# Autodesk Inventor assembly: A2017_T5_08
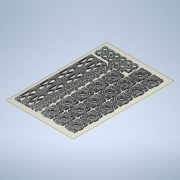
[picture p0: Inventor's stored thumbnail of the model, 180x180]
Saved by Autodesk Inventor 2022 (Build 260153000, 153)
## iProperties
Created: 2022-09-28
Part Number: A2017_T5_08
Document SubType Name: Assembly
Designer: Masato
Author: Masato
## Documents named in this file (6)
- C:\Users\ヨコオリク\Documents\CITBrains\SUSTAINA-OP\Cam\A2017_T5\A2017_T5_08.iam
- C:\Users\ヨコオリク\Documents\CITBrains\SUSTAINA-OP\Cam\DisposableBoard.ipt
- C:\Users\ヨコオリク\Documents\CITBrains\SUSTAINA-OP\UpperBody\UpperBody_horn_frame.ipt
- C:\Users\ヨコオリク\Documents\CITBrains\SUSTAINA-OP\LowerBody\Foot\Foot_root_block.ipt
- C:\Users\ヨコオリク\Documents\CITBrains\SUSTAINA-OP\LowerBody\Knee\Knee_clamp.ipt
- C:\Users\ヨコオリク\Documents\CITBrains\SUSTAINA-OP\LowerBody\Link\BackLink_diagonal.ipt
## Components (61 placed, 5 different names)
1. DisposableBoard:1 — フラッシュ:1, フラッシュ:2, フラッシュ:3, フラッシュ:4, Flush:5, 正接:1, フラッシュ:8, フラッシュ:9, フラッシュ:10, フラッシュ:11, 正接:6
2. Foot_root_block:33 — メイト:14, メイト:15, メイト:16
3. UpperBody_horn_frame:1 — Mate:3, Flush:5, 正接:5
4. UpperBody_horn_frame:2
5. UpperBody_horn_frame:3
6. UpperBody_horn_frame:4
7. UpperBody_horn_frame:5
8. UpperBody_horn_frame:6
9. UpperBody_horn_frame:7 — 正接:1
10. UpperBody_horn_frame:8
11. UpperBody_horn_frame:9
12. UpperBody_horn_frame:10
13. UpperBody_horn_frame:11
14. UpperBody_horn_frame:12
15. UpperBody_horn_frame:13 — メイト:6, フラッシュ:8, 正接:5
16. UpperBody_horn_frame:14
17. UpperBody_horn_frame:15
18. UpperBody_horn_frame:16
19. UpperBody_horn_frame:17 — メイト:16
20. BackLink_diagonal:1 — メイト:7, フラッシュ:9, フラッシュ:10
21. BackLink_diagonal:2 — メイト:10
22. BackLink_diagonal:3
23. BackLink_diagonal:4
24. BackLink_diagonal:5
25. BackLink_diagonal:6
26. BackLink_diagonal:7 — 正接:7
27. BackLink_diagonal:8 — メイト:12
28. Foot_root_block:11 — メイト:9, フラッシュ:11, メイト:10
29. Foot_root_block:12
30. Foot_root_block:13
31. Foot_root_block:14
32. Foot_root_block:15
33. Foot_root_block:16
34. Foot_root_block:17
35. Foot_root_block:18
36. Foot_root_block:19
37. Foot_root_block:20
38. Foot_root_block:21
39. Foot_root_block:22
40. Foot_root_block:23
41. Foot_root_block:24
42. Foot_root_block:25
43. Foot_root_block:26
44. Foot_root_block:27
45. Foot_root_block:28
46. Foot_root_block:29
47. Foot_root_block:30 — メイト:13
48. Knee_clamp:1 — メイト:8, 角度:1, 正接:6, 正接:7
49. Knee_clamp:2
50. Knee_clamp:3
51. Knee_clamp:4
52. Knee_clamp:5
53. Knee_clamp:6
54. Knee_clamp:7
55. Knee_clamp:8
56. Knee_clamp:9
57. Knee_clamp:10
58. Knee_clamp:11
59. Knee_clamp:12
60. Foot_root_block:31 — メイト:11, メイト:12, メイト:13
61. Foot_root_block:32 — メイト:15
## Component patterns: (12 elements, first: UpperBody_horn_frame:1), (5 elements, first: UpperBody_horn_frame:13), (8 elements, first: BackLink_diagonal:1), (20 elements, first: Foot_root_block:11), (12 elements, first: Knee_clamp:1), (2 elements, first: Foot_root_block:31)
## Relationships (26: Mate 12, Flush 9, Tangent 4, Angle 1)
- フラッシュ:1 [Flush]: DisposableBoard:1
- フラッシュ:2 [Flush]: DisposableBoard:1
- フラッシュ:3 [Flush]: DisposableBoard:1
- フラッシュ:4 [Flush]: DisposableBoard:1
- Mate:3: UpperBody_horn_frame:1
- Flush:5 (-2 mm): DisposableBoard:1 ↔ UpperBody_horn_frame:1
- メイト:6 [Mate]: UpperBody_horn_frame:13
- 正接:1 [Tangent] (2.1 mm): DisposableBoard:1 ↔ UpperBody_horn_frame:7
- フラッシュ:8 [Flush] (2 mm): DisposableBoard:1 ↔ UpperBody_horn_frame:13
- メイト:7 [Mate]: BackLink_diagonal:1
- フラッシュ:9 [Flush] (2 mm): DisposableBoard:1 ↔ BackLink_diagonal:1
- フラッシュ:10 [Flush] (2 mm): DisposableBoard:1 ↔ BackLink_diagonal:1
- メイト:8 [Mate]: Knee_clamp:1
- 角度:1 [Angle] (45 deg): Knee_clamp:1
- 正接:5 [Tangent] (2.1 mm): UpperBody_horn_frame:1 ↔ UpperBody_horn_frame:13
- メイト:9 [Mate]: Foot_root_block:11
- フラッシュ:11 [Flush] (2 mm): DisposableBoard:1 ↔ Foot_root_block:11
- メイト:10 [Mate] (2.1 mm): BackLink_diagonal:2 ↔ Foot_root_block:11
- 正接:6 [Tangent] (2 mm): DisposableBoard:1 ↔ Knee_clamp:1
- 正接:7 [Tangent] (11.1 mm): BackLink_diagonal:7 ↔ Knee_clamp:1
- メイト:11 [Mate]: Foot_root_block:31
- メイト:12 [Mate] (2.1 mm): BackLink_diagonal:8 ↔ Foot_root_block:31
- メイト:13 [Mate] (2.1 mm): Foot_root_block:30 ↔ Foot_root_block:31
- メイト:14 [Mate]: Foot_root_block:33
- メイト:15 [Mate] (2.1 mm): Foot_root_block:33 ↔ Foot_root_block:32
- メイト:16 [Mate] (2.1 mm): Foot_root_block:33 ↔ UpperBody_horn_frame:17
